# Autodesk Inventor assembly: asse_s_tstage
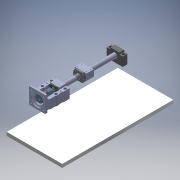
[picture p0: Inventor's stored thumbnail of the model, 180x180]
Saved by Autodesk Inventor 2019 (Build 230136000, 136)
## iProperties
Created: 2022-09-02
Part Number: asse_s_tstage
Document SubType Name: Assembly
Designer: kananovicha
Author: kananovicha
## Documents named in this file (4)
- C:\Users\kananovicha\OneDrive\work\workAppState\prj_shocksL\s_tstage\drawingsGit\s_tstage\asse_s_tstage\asse_s_tstage.iam
- C:\Users\kananovicha\OneDrive\work\workAppState\prj_shocksL\s_tstage\drawingsGit\s_tstage\mplate\mplate.ipt
- C:\Users\kananovicha\OneDrive\work\workAppState\prj_shocksL\s_tstage\drawingsGit\s_tstage\3rdParty\ballScrewAssembly\2510 L=400.iam
- C:\Users\kananovicha\OneDrive\work\workAppState\prj_shocksL\s_tstage\drawingsGit\s_tstage\allmainparams\allmainparams.ipt
## Components (2 placed, 2 different names)
1. mplate:1 — Flush:1
2. 2510 L=400:1 [sub-assembly] — Flush:1
## Relationships (1: Flush 1)
- Flush:1 (104.9 mm): mplate:1 ↔ 2510 L=400:1
## Named parameters: asse_sfu_offset_wid = 104.9 mm
